# Autodesk Inventor assembly: DopelZahnrad
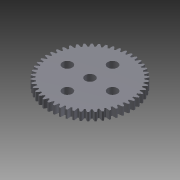
[picture p0: Inventor's stored thumbnail of the model, 180x180]
Saved by Autodesk Inventor 2014 (Build 180170000, 170)
## iProperties
Created: 2013-05-31
Part Number: DopelZahnrad
Document SubType Name: Assembly
Designer: hanse
Author: hanse
## Documents named in this file (3)
- C:\Users\hanse\Desktop\Beep\Hardware\GetriebeB\DoppelZahnrad.iam
- C:\Users\hanse\Desktop\Beep\Hardware\GetriebeB\DopelZahnrad\Konstruktions-Assistent\Stirnräder3.iam
- C:\Users\hanse\Desktop\Beep\Hardware\GetriebeB\DopelZahnrad\Konstruktions-Assistent\Stirnräder1.iam
## Components (2 placed, 1 different names)
1. Stirnräder:2 [sub-assembly] — Passend:2, Passend:4, Passend:7
2. Stirnräder:3 [sub-assembly] — Passend:3, Passend:4, Passend:5
## Relationships (6: Mate 6)
- Passend:2 [Mate]: Stirnräder:2
- Passend:3 [Mate]: Stirnräder:3
- Passend:4 [Mate]: Stirnräder:2 ↔ Stirnräder:3
- Passend:5 [Mate]: Stirnräder:3
- Passend:6 [Mate]
- Passend:7 [Mate]: Stirnräder:2
